# Autodesk Inventor assembly: case_assembly
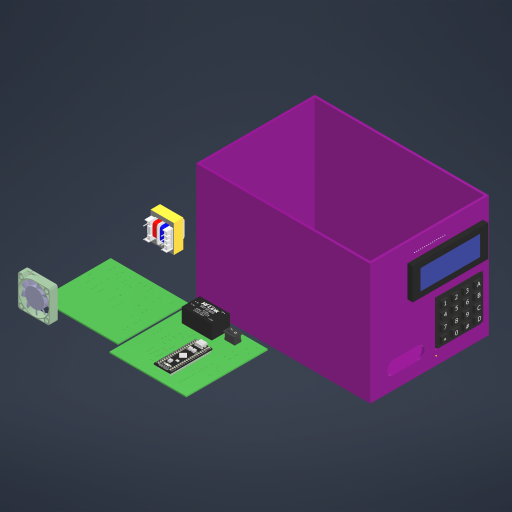
[picture p0: Inventor's stored thumbnail of the model, 512x512]
Saved by Autodesk Inventor 2023 (Build 270158000, 158)
## iProperties
Created: 2022-11-26
Part Number: case_assembly
Document SubType Name: Assembly
Designer: washington
Author: washington
## Documents named in this file (8)
- C:\Users\washi\Desktop\FYP18-22\ELECTRONICS_CAD\case_assembly.iam
- C:\Users\washi\Desktop\FYP18-22\ELECTRONICS_CAD\perspex_shell\perspex_shell.ipt
- C:\Users\washi\Desktop\FYP18-22\ELECTRONICS_CAD\pcbs\Electronic design.iam
- C:\Users\washi\Desktop\FYP18-22\ELECTRONICS_CAD\transformer\Transformer EI35 12V150mA 2+4.iam
- C:\Users\washi\Desktop\FYP18-22\ELECTRONICS_CAD\keypad\keypad 4x4.ipt
- C:\Users\washi\Desktop\FYP18-22\ELECTRONICS_CAD\fan\DC Brushless fan JIESAMMY 40x40x25 12V 1.2W.iam
- C:\Users\washi\Desktop\FYP18-22\ELECTRONICS_CAD\pcbs\triac_pcb\TRIAC_SWITCHING.iam
- C:\Users\washi\Desktop\FYP18-22\ELECTRONICS_CAD\lcd\LCD_I2C\Lcd i2c.iam
## Components (7 placed, 7 different names)
1. perspex_shell:1 — Mate:5, Mate:6, Mate:7, Mate:8, Mate:9, Mate:10
2. Electronic design:1 [sub-assembly]
3. Transformer EI35 12V150mA 2+4:1 [sub-assembly]
4. keypad 4x4:1 — Mate:5, Mate:6, Mate:10
5. DC Brushless fan JIESAMMY 40x40x25 12V 1.2W:1 [sub-assembly]
6. TRIAC_SWITCHING:1 [sub-assembly]
7. Lcd i2c:1 [sub-assembly] — Mate:7, Mate:8, Mate:9
## Relationships (6: Mate 6)
- Mate:5: perspex_shell:1 ↔ keypad 4x4:1
- Mate:6: perspex_shell:1 ↔ keypad 4x4:1
- Mate:7: perspex_shell:1 ↔ Lcd i2c:1
- Mate:8: perspex_shell:1 ↔ Lcd i2c:1
- Mate:9: perspex_shell:1 ↔ Lcd i2c:1
- Mate:10: perspex_shell:1 ↔ keypad 4x4:1
